# Autodesk Inventor assembly: 21-092-PHANTOM-HRDSET
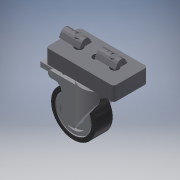
[picture p0: Inventor's stored thumbnail of the model, 180x180]
Saved by Autodesk Inventor 2018 (Build 220105000, 105)
## iProperties
Created: 2004-11-19
Part Number: 21-092-PHANTOM-HRDSET
Document SubType Name: Assembly
Designer: Autodesk, Inc.
Manufacturer: Standard
Standards Organization: Custom
Description: PHANTOM, CASTER, LOCKING, HARDWARE SET
Catalog Web Link: http://www.parker.com/ead/cm1.asp?cmid=809
Vendor: PARKER IPS
Mass: 442.443 g
Surface Area: 373.841 cm^2
Volume: 105.266 cm^3
Density: 4.20308 g/cm^3
CAGE: 1LJX3
Dept. ID: Product Design
Description #2: ---
Finish #1: ---
Finish #2: ---
Material ID: ---
Project Number: ---
Author: Autodesk, Inc.
## Documents named in this file (4)
- C:\Autodesk\autodesk_inventor_2017_samples\Models\Assemblies\Test Station\Components\21-092 Caster Phantom.iam
- C:\Autodesk\autodesk_inventor_2017_samples\Models\Assemblies\Test Station\Components\21-092 Caster.ipt
- C:\Autodesk\autodesk_inventor_2017_samples\Models\Assemblies\Test Station\Components\21-09x_Caster_Mnt_Phantom.iam
- C:\Autodesk\autodesk_inventor_2017_samples\Models\Assemblies\Test Station\Components\M10x25-Spring Phantom.iam
## Components (3 placed, 3 different names)
1. 21-092 Caster:1
2. 21-09x_Caster_Mnt_Phantom:1 [sub-assembly]
3. M10x25-Spring Phantom:1 [sub-assembly]
## Relationships (2: Insert 2)
- [Insert]: 21-092 Caster:1 ↔ M10x25-Spring Phantom:1
- [Insert]: 21-092 Caster:1 ↔ 21-09x_Caster_Mnt_Phantom:1
